# Autodesk Inventor assembly: Platten mit Verbindungen und Rahmen
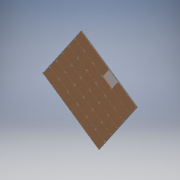
[picture p0: Inventor's stored thumbnail of the model, 180x180]
Saved by Autodesk Inventor 2019.5 (Build 235369000, 369)
## iProperties
Created: 2021-09-27
Part Number: Platten mit Verbindungen und Rahmen
Material: Generisch
Document SubType Name: Assembly
Designer: mritt
Author: mritt
## Documents named in this file (4)
- D:\Studium\Universität Stuttgart\Sonstige Tätigkeiten\Tätigkeit_studentische_Hilfskraft_Informatik\Hiwi-Projekt\CAD-Dateien\Arena\Arena Rescue\Platten mit Verbindungen und Rahmen.iam
- D:\Studium\Universität Stuttgart\Sonstige Tätigkeiten\Tätigkeit_studentische_Hilfskraft_Informatik\Hiwi-Projekt\CAD-Dateien\Arena\Arena Rescue\Bauteil3.ipt
- D:\Studium\Universität Stuttgart\Sonstige Tätigkeiten\Tätigkeit_studentische_Hilfskraft_Informatik\Hiwi-Projekt\CAD-Dateien\Arena\Arena Rescue\Rahmen.ipt
- D:\Studium\Universität Stuttgart\Sonstige Tätigkeiten\Tätigkeit_studentische_Hilfskraft_Informatik\Hiwi-Projekt\CAD-Dateien\Arena\Arena Rescue\Bauteil2.ipt
## Components (65 placed, 3 different names)
1. Bauteil3:3 — Fluchtend:1, Fluchtend:3, Fluchtend:4, Passend:1, Fluchtend:16, Passend:66, Passend:140
2. Bauteil3:6 — Fluchtend:1, Fluchtend:8, Passend:54, Passend:55, Passend:66, Passend:67, Fluchtend:90
3. Bauteil3:7 — Fluchtend:3, Passend:65, Fluchtend:39
4. Bauteil3:8 — Passend:61, Passend:62, Passend:134
5. Rahmen:1 — Fluchtend:4, Passend:1, Passend:67, Passend:137
6. Bauteil3:9 — Fluchtend:8, Passend:63, Passend:64, Passend:73, Fluchtend:50, Passend:76, Fluchtend:51
7. Bauteil2:6 — Passend:45, Fluchtend:34, Fluchtend:38
8. Bauteil3:14 — Fluchtend:16, Passend:21, Fluchtend:37, Fluchtend:38, Passend:58, Passend:61
9. Bauteil2:7 — Fluchtend:34, Fluchtend:35, Fluchtend:36
10. Bauteil2:8 — Passend:21, Fluchtend:35, Passend:59, Passend:60
11. Bauteil3:15 — Fluchtend:17, Fluchtend:36, Fluchtend:42, Passend:144
12. Bauteil3:16 — Fluchtend:17
13. Bauteil2:9 — Passend:55
14. Bauteil2:10 — Fluchtend:28, Fluchtend:31
15. Bauteil3:17 — Passend:54, Fluchtend:39, Passend:74, Passend:84
16. Bauteil3:18 — Fluchtend:27, Passend:48, Fluchtend:31, Passend:65, Passend:138
17. Bauteil3:19 — Fluchtend:26, Passend:49, Passend:56, Passend:57, Passend:60
18. Bauteil2:11 — Passend:48
19. Bauteil2:12 — Fluchtend:28, Passend:49, Passend:64
20. Bauteil3:20 — Fluchtend:27, Passend:63, Fluchtend:46, Passend:75, Fluchtend:89
21. Bauteil3:21 — Fluchtend:26, Passend:56, Passend:59, Passend:139
22. Bauteil2:13 — Fluchtend:40
23. Bauteil2:14 — Fluchtend:40, Fluchtend:42
24. Bauteil3:22 — Passend:45, Fluchtend:37, Passend:58, Passend:137
25. Bauteil3:23 — Passend:57, Passend:62
26. Bauteil2:15 — Passend:76
27. Bauteil2:16 — Passend:79, Passend:80
28. Bauteil3:24 — Fluchtend:46, Passend:72, Passend:74, Passend:75, Fluchtend:52, Fluchtend:54, Passend:81
29. Bauteil2:17 — Passend:110, Passend:111
30. Bauteil2:18 — Passend:78
31. Bauteil3:25 — Passend:72, Passend:73, Fluchtend:50, Fluchtend:53, Passend:77, Fluchtend:55
32. Bauteil2:19 — Passend:81, Passend:82, Passend:83
33. Bauteil2:23 — Passend:86, Passend:88, Passend:91, Passend:95, Fluchtend:90
34. Bauteil2:26 — Passend:84, Passend:85, Passend:87
35. Bauteil3:27 — Fluchtend:51, Passend:87, Passend:88
36. Bauteil3:28 — Fluchtend:52, Passend:77, Passend:78, Passend:80, Passend:101, Fluchtend:67, Fluchtend:68
37. Bauteil3:29 — Passend:142, Fluchtend:91, Passend:145
38. Bauteil3:30 — Fluchtend:53, Passend:138, Passend:139, Passend:141, Fluchtend:91, Fluchtend:92, Passend:143
39. Bauteil3:31 — Fluchtend:54, Passend:79, Passend:82, Passend:100, Fluchtend:70
40. Bauteil3:32 — Fluchtend:55, Passend:83, Passend:85, Passend:86, Passend:94
41. Bauteil2:27
42. Bauteil3:34 — Passend:91
43. Bauteil2:28 — Fluchtend:57, Passend:94, Passend:99
44. Bauteil3:35 — Fluchtend:57, Passend:95, Fluchtend:59, Fluchtend:70
45. Bauteil2:29 — Fluchtend:60, Passend:100
46. Bauteil3:36 — Passend:99, Fluchtend:59, Fluchtend:60, Fluchtend:61
47. Bauteil2:30 — Passend:101, Passend:109, Passend:130
48. Bauteil3:37 — Fluchtend:61, Fluchtend:69
49. Bauteil3:38 — Passend:110
50. Bauteil2:31 — Passend:135, Passend:136
51. Bauteil2:32 — Passend:131
52. Bauteil3:39 — Fluchtend:67, Passend:111, Fluchtend:88
53. Bauteil3:40 — Fluchtend:68, Passend:109
54. Bauteil2:33 — Passend:129
55. Bauteil3:41 — Fluchtend:69, Passend:130, Fluchtend:86
56. Bauteil2:34
57. Bauteil2:35
58. Bauteil3:43 — Fluchtend:84, Passend:131
59. Bauteil3:44 — Passend:129, Fluchtend:84, Fluchtend:85, Fluchtend:86
60. Bauteil2:36 — Fluchtend:85
61. Bauteil3:49 — Passend:140, Passend:141, Fluchtend:89, Passend:142
62. Bauteil2:38 — Passend:134
63. Bauteil3:50 — Passend:136
64. Bauteil3:51 — Fluchtend:88, Passend:135
65. Bauteil3:52 — Fluchtend:92, Passend:143, Passend:144, Passend:145
## Relationships (176: Mate 109, Flush 67)
- Fluchtend:1 [Flush]: Bauteil3:3 ↔ Bauteil3:6
- [Flush]: Bauteil3:7 ↔ Bauteil3:8
- Fluchtend:3 [Flush]: Bauteil3:3 ↔ Bauteil3:7
- Fluchtend:4 [Flush]: Bauteil3:3 ↔ Rahmen:1
- Passend:1 [Mate]: Bauteil3:3 ↔ Rahmen:1
- Fluchtend:8 [Flush]: Bauteil3:6 ↔ Bauteil3:9
- [Mate]: Bauteil2:6 ↔ Bauteil3:14
- [Flush]: Bauteil2:7 ↔ Bauteil2:8
- [Mate]: Bauteil2:7 ↔ Bauteil3:15
- [Mate]: Bauteil3:15 ↔ Bauteil3:16
- [Mate]: Bauteil2:7 ↔ Bauteil3:16
- [Mate]: Bauteil2:8 ↔ Bauteil3:16
- [Mate]: Bauteil2:8 ↔ Bauteil3:15
- Fluchtend:16 [Flush]: Bauteil3:3 ↔ Bauteil3:14
- Fluchtend:17 [Flush]: Bauteil3:15 ↔ Bauteil3:16
- Passend:21 [Mate]: Bauteil3:14 ↔ Bauteil2:8
- [Flush]: Bauteil3:17 ↔ Bauteil3:19
- [Flush]: Bauteil3:18 ↔ Bauteil3:19
- [Flush]: Bauteil2:9 ↔ Bauteil2:10
- [Mate]: Bauteil2:9 ↔ Bauteil3:17
- [Mate]: Bauteil3:17 ↔ Bauteil3:18
- [Mate]: Bauteil2:9 ↔ Bauteil3:18
- [Mate]: Bauteil2:10 ↔ Bauteil3:18
- [Mate]: Bauteil2:10 ↔ Bauteil3:17
- [Flush]: Bauteil2:11 ↔ Bauteil2:12
- [Mate]: Bauteil2:11 ↔ Bauteil3:20
- [Mate]: Bauteil3:20 ↔ Bauteil3:21
- [Mate]: Bauteil2:11 ↔ Bauteil3:21
- [Mate]: Bauteil2:12 ↔ Bauteil3:21
- [Mate]: Bauteil2:12 ↔ Bauteil3:20
- [Flush]: Bauteil2:13 ↔ Bauteil2:14
- [Mate]: Bauteil2:13 ↔ Bauteil3:22
- [Mate]: Bauteil3:22 ↔ Bauteil3:23
- [Mate]: Bauteil2:13 ↔ Bauteil3:23
- [Mate]: Bauteil2:14 ↔ Bauteil3:23
- [Mate]: Bauteil2:14 ↔ Bauteil3:22
- [Mate]: Bauteil3:18 ↔ Bauteil2:11
- [Mate]: Bauteil2:10 ↔ Bauteil3:20
- [Flush]: Bauteil3:22 ↔ Bauteil3:23
- [Flush]: Bauteil3:18 ↔ Bauteil3:22
- [Mate]: Bauteil2:11 ↔ Bauteil3:22
- [Mate]: Bauteil3:21 ↔ Bauteil2:14
- [Mate]: Bauteil3:19 ↔ Bauteil2:14
- Fluchtend:26 [Flush]: Bauteil3:19 ↔ Bauteil3:21
- Fluchtend:27 [Flush]: Bauteil3:18 ↔ Bauteil3:20
- Fluchtend:28 [Flush]: Bauteil2:10 ↔ Bauteil2:12
- Passend:45 [Mate]: Bauteil2:6 ↔ Bauteil3:22
- Passend:48 [Mate]: Bauteil3:18 ↔ Bauteil2:11
- Fluchtend:31 [Flush]: Bauteil2:10 ↔ Bauteil3:18
- Passend:49 [Mate]: Bauteil3:19 ↔ Bauteil2:12
- Fluchtend:34 [Flush]: Bauteil2:6 ↔ Bauteil2:7
- Fluchtend:35 [Flush]: Bauteil2:7 ↔ Bauteil2:8
- Fluchtend:36 [Flush]: Bauteil2:7 ↔ Bauteil3:15
- Fluchtend:37 [Flush]: Bauteil3:14 ↔ Bauteil3:22
- Fluchtend:38 [Flush]: Bauteil2:6 ↔ Bauteil3:14
- Passend:54 [Mate]: Bauteil3:6 ↔ Bauteil3:17
- Passend:55 [Mate]: Bauteil3:6 ↔ Bauteil2:9
- Passend:56 [Mate]: Bauteil3:19 ↔ Bauteil3:21
- Passend:57 [Mate]: Bauteil3:19 ↔ Bauteil3:23
- Passend:58 [Mate]: Bauteil3:14 ↔ Bauteil3:22
- Passend:59 [Mate]: Bauteil2:8 ↔ Bauteil3:21
- Passend:60 [Mate]: Bauteil2:8 ↔ Bauteil3:19
- Passend:61 [Mate]: Bauteil3:8 ↔ Bauteil3:14
- Passend:62 [Mate]: Bauteil3:8 ↔ Bauteil3:23
- Passend:63 [Mate]: Bauteil3:9 ↔ Bauteil3:20
- Passend:64 [Mate]: Bauteil3:9 ↔ Bauteil2:12
- Passend:65 [Mate]: Bauteil3:7 ↔ Bauteil3:18
- Fluchtend:39 [Flush]: Bauteil3:7 ↔ Bauteil3:17
- Fluchtend:40 [Flush]: Bauteil2:13 ↔ Bauteil2:14
- Fluchtend:42 [Flush]: Bauteil3:15 ↔ Bauteil2:14
- Passend:66 [Mate]: Bauteil3:3 ↔ Bauteil3:6
- Passend:67 [Mate]: Bauteil3:6 ↔ Rahmen:1
- [Flush]: Bauteil2:15 ↔ Bauteil2:16
- [Mate]: Bauteil2:15 ↔ Bauteil3:24
- [Mate]: Bauteil2:16 ↔ Bauteil3:24
- [Flush]: Bauteil2:15 ↔ Bauteil2:16
- [Flush]: Bauteil2:15 ↔ Bauteil3:24
- Fluchtend:46 [Flush]: Bauteil3:20 ↔ Bauteil3:24
- [Flush]: Bauteil2:17 ↔ Bauteil2:18
- [Mate]: Bauteil2:17 ↔ Bauteil3:25
- [Mate]: Bauteil2:18 ↔ Bauteil3:25
- [Flush]: Bauteil2:17 ↔ Bauteil2:18
- [Flush]: Bauteil2:17 ↔ Bauteil3:25
- Passend:72 [Mate]: Bauteil3:24 ↔ Bauteil3:25
- Passend:73 [Mate]: Bauteil3:9 ↔ Bauteil3:25
- Passend:74 [Mate]: Bauteil3:17 ↔ Bauteil3:24
- Passend:75 [Mate]: Bauteil3:20 ↔ Bauteil3:24
- Fluchtend:50 [Flush]: Bauteil3:9 ↔ Bauteil3:25
- Passend:76 [Mate]: Bauteil3:9 ↔ Bauteil2:15
- Fluchtend:51 [Flush]: Bauteil3:9 ↔ Bauteil3:27
- Fluchtend:52 [Flush]: Bauteil3:24 ↔ Bauteil3:28
- Fluchtend:53 [Flush]: Bauteil3:25 ↔ Bauteil3:30
- Passend:77 [Mate]: Bauteil3:25 ↔ Bauteil3:28
- Passend:78 [Mate]: Bauteil2:18 ↔ Bauteil3:28
- Fluchtend:54 [Flush]: Bauteil3:24 ↔ Bauteil3:31
- Fluchtend:55 [Flush]: Bauteil3:25 ↔ Bauteil3:32
- Passend:79 [Mate]: Bauteil2:16 ↔ Bauteil3:31
- Passend:80 [Mate]: Bauteil2:16 ↔ Bauteil3:28
- Passend:81 [Mate]: Bauteil3:24 ↔ Bauteil2:19
- Passend:82 [Mate]: Bauteil2:19 ↔ Bauteil3:31
- Passend:83 [Mate]: Bauteil2:19 ↔ Bauteil3:32
- Passend:84 [Mate]: Bauteil3:17 ↔ Bauteil2:26
- Passend:85 [Mate]: Bauteil2:26 ↔ Bauteil3:32
- Passend:86 [Mate]: Bauteil2:23 ↔ Bauteil3:32
- Passend:87 [Mate]: Bauteil2:26 ↔ Bauteil3:27
- Passend:88 [Mate]: Bauteil2:23 ↔ Bauteil3:27
- [Mate]: Bauteil2:27 ↔ Bauteil3:34
- [Flush]: Bauteil2:27 ↔ Bauteil3:34
- Passend:91 [Mate]: Bauteil2:23 ↔ Bauteil3:34
- [Mate]: Bauteil2:28 ↔ Bauteil3:35
- Fluchtend:57 [Flush]: Bauteil2:28 ↔ Bauteil3:35
- Passend:94 [Mate]: Bauteil3:32 ↔ Bauteil2:28
- Passend:95 [Mate]: Bauteil2:23 ↔ Bauteil3:35
- [Mate]: Bauteil2:29 ↔ Bauteil3:36
- [Mate]: Bauteil2:30 ↔ Bauteil3:37
- [Flush]: Bauteil2:30 ↔ Bauteil3:37
- [Mate]: Bauteil2:29 ↔ Bauteil3:37
- Passend:99 [Mate]: Bauteil2:28 ↔ Bauteil3:36
- Fluchtend:59 [Flush]: Bauteil3:35 ↔ Bauteil3:36
- Fluchtend:60 [Flush]: Bauteil2:29 ↔ Bauteil3:36
- Fluchtend:61 [Flush]: Bauteil3:36 ↔ Bauteil3:37
- Passend:100 [Mate]: Bauteil3:31 ↔ Bauteil2:29
- Passend:101 [Mate]: Bauteil3:28 ↔ Bauteil2:30
- [Flush]: Bauteil2:31 ↔ Bauteil2:32
- [Mate]: Bauteil2:31 ↔ Bauteil3:39
- [Mate]: Bauteil2:32 ↔ Bauteil3:39
- [Flush]: Bauteil2:31 ↔ Bauteil2:32
- [Flush]: Bauteil2:31 ↔ Bauteil3:39
- [Mate]: Bauteil3:38 ↔ Bauteil3:39
- [Flush]: Bauteil3:38 ↔ Bauteil3:39
- [Mate]: Bauteil3:39 ↔ Bauteil3:40
- [Mate]: Bauteil2:32 ↔ Bauteil3:40
- [Mate]: Bauteil2:33 ↔ Bauteil3:41
- [Flush]: Bauteil2:33 ↔ Bauteil3:41
- [Mate]: Bauteil3:40 ↔ Bauteil2:33
- Fluchtend:67 [Flush]: Bauteil3:28 ↔ Bauteil3:39
- Fluchtend:68 [Flush]: Bauteil3:28 ↔ Bauteil3:40
- Fluchtend:69 [Flush]: Bauteil3:37 ↔ Bauteil3:41
- Fluchtend:70 [Flush]: Bauteil3:31 ↔ Bauteil3:35
- Passend:109 [Mate]: Bauteil2:30 ↔ Bauteil3:40
- Passend:110 [Mate]: Bauteil2:17 ↔ Bauteil3:38
- Passend:111 [Mate]: Bauteil2:17 ↔ Bauteil3:39
- [Flush]: Bauteil2:34 ↔ Bauteil2:35
- [Mate]: Bauteil2:34 ↔ Bauteil3:43
- [Mate]: Bauteil2:35 ↔ Bauteil3:43
- [Flush]: Bauteil2:34 ↔ Bauteil2:35
- [Flush]: Bauteil2:34 ↔ Bauteil3:43
- [Mate]: Bauteil3:43 ↔ Bauteil3:44
- [Mate]: Bauteil2:35 ↔ Bauteil3:44
- [Mate]: Bauteil3:44 ↔ Bauteil2:36
- Passend:129 [Mate]: Bauteil2:33 ↔ Bauteil3:44
- Passend:130 [Mate]: Bauteil2:30 ↔ Bauteil3:41
- Fluchtend:84 [Flush]: Bauteil3:43 ↔ Bauteil3:44
- Fluchtend:85 [Flush]: Bauteil3:44 ↔ Bauteil2:36
- Fluchtend:86 [Flush]: Bauteil3:41 ↔ Bauteil3:44
- Passend:131 [Mate]: Bauteil2:32 ↔ Bauteil3:43
- [Mate]: Bauteil3:50 ↔ Bauteil3:51
- [Flush]: Bauteil3:50 ↔ Bauteil3:51
- [Mate]: Bauteil2:38 ↔ Bauteil3:50
- Fluchtend:88 [Flush]: Bauteil3:39 ↔ Bauteil3:51
- Passend:134 [Mate]: Bauteil3:8 ↔ Bauteil2:38
- Passend:135 [Mate]: Bauteil2:31 ↔ Bauteil3:51
- Passend:136 [Mate]: Bauteil2:31 ↔ Bauteil3:50
- Passend:137 [Mate]: Rahmen:1 ↔ Bauteil3:22
- Passend:138 [Mate]: Bauteil3:18 ↔ Bauteil3:30
- Passend:139 [Mate]: Bauteil3:21 ↔ Bauteil3:30
- Passend:140 [Mate]: Bauteil3:3 ↔ Bauteil3:49
- Passend:141 [Mate]: Bauteil3:30 ↔ Bauteil3:49
- Fluchtend:89 [Flush]: Bauteil3:20 ↔ Bauteil3:49
- Passend:142 [Mate]: Bauteil3:29 ↔ Bauteil3:49
- Fluchtend:90 [Flush]: Bauteil3:6 ↔ Bauteil2:23
- Fluchtend:91 [Flush]: Bauteil3:29 ↔ Bauteil3:30
- Fluchtend:92 [Flush]: Bauteil3:30 ↔ Bauteil3:52
- Passend:143 [Mate]: Bauteil3:30 ↔ Bauteil3:52
- Passend:144 [Mate]: Bauteil3:15 ↔ Bauteil3:52
- Passend:145 [Mate]: Bauteil3:29 ↔ Bauteil3:52
## Named parameters: d1_d0 = 0 mm, d22_d20 = 0 mm, d28_d20 = 0 mm, d29_d21 = 0 mm, d30_d12 = 0 mm, d31_d15 = 0 mm, d32_d16 = 0 mm, d33_d17 = 0 mm, d43_d37 = 0 mm, d44_d38 = 0 mm, d45_d39 = 0 mm, d46_d40 = 0 mm, d47_d41 = 0 mm, d48_d42 = 0 mm, d49_d20 = 0 mm, d50_d21 = 0 mm, d51_d22_d20 = 0 mm, d52_d23_d21 = 0 mm, d53_d24_d12 = 0 mm, d54_d25_d15 = 0 mm, d55_d26_d16 = 0 mm, d56_d27_d17 = 0 mm, d57_d28_d20 = 0 mm, d58_d29_d21 = 0 mm, d59_d30_d12 = 0 mm, d60_d31_d15 = 0 mm, d61_d32_d16 = 0 mm, d62_d33_d17 = 0 mm, d63_d36 = 0 mm, d64_d6 = 0 mm, d65_d8 = 0 mm, d66_d12 = 0 mm, d67_d15 = 0 mm, d68_d16 = 0 mm, d69_d17 = 0 mm, d118_d29_d21 = 0 mm, d119_d30_d12 = 0 mm, d120_d31_d15 = 0 mm, d121_d93 = 0 mm, d122_d94 = 0 mm, d124_d118_d29_d21 = 0 mm, d125_d119_d30_d12 = 0 mm, d126_d120_d31_d15 = 0 mm, d127_d121_d93 = 0 mm, d128_d122_d94 = 0 mm, d152_d96 = 0 mm, d154_d22_d20 = 0 mm, d156_d155 = 0 mm, d161_d160 = 0 mm, d162_d155 = 0 mm, d163_d156_d155 = 0 mm, d164_d158 = 0 mm, d171_d163_d156_d155 = 0 mm, d172_d164_d158 = 0 mm, d173_d170 = 0 mm, d174_d138 = 0 mm, d175_d139 = 0 mm, d176_d124_d118_d29_d21 = 0 mm, d177_d125_d119_d30_d12 = 0 mm, d178_d126_d120_d31_d15 = 0 mm, d179_d127_d121_d93 = 0 mm, d180_d128_d122_d94 = 0 mm, d181_d130 = 0 mm, d182_d133 = 0 mm, d196_d170 = 0 mm, d211_d138 = 0 mm, d212_d139 = 0 mm, d213_d124_d118_d29_d21 = 0 mm, d214_d125_d119_d30_d12 = 0 mm, d215_d126_d120_d31_d15 = 0 mm, d216_d127_d121_d93 = 0 mm, d217_d128_d122_d94 = 0 mm, d227_d226 = 0 mm, d228_d222 = 0 mm, d229_d211_d138 = 0 mm
